# Autodesk Inventor assembly: Base_Rotation
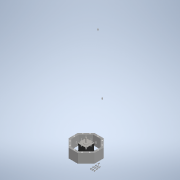
[picture p0: Inventor's stored thumbnail of the model, 180x180]
Saved by Autodesk Inventor 2022 (Build 260153000, 153)
## iProperties
Created: 2022-03-21
Part Number: Base_Rotation
Document SubType Name: Assembly
Designer: Mlees
Author: Mlees
## Documents named in this file (7)
- C:\Users\Mlees\Desktop\504Engineering\Project_0000\Designs\Design_1\Base_Rotation.iam
- C:\Users\Mlees\Desktop\504Engineering\Project_0000\Designs\Design_1\Created_Parts\Base_Mount.ipt
- C:\Users\Mlees\Desktop\504Engineering\Stepper-Servo_Based_Robotic_Arm\Designs\Version_8\Downloaded_Parts\Nema_17\Nema 17.ipt
- C:\Users\Mlees\Desktop\504Engineering\Project_0000\Designs\Design_1\Created_Parts\Base_Lid.ipt
- C:\Users\Mlees\Desktop\504Engineering\Project_0000\Designs\Design_1\Downloaded_Parts\Stainless Steel Pan Head Phillips Screws_m2.5x8mm.ipt
- C:\Users\Mlees\Desktop\504Engineering\Project_0000\Designs\Design_1\Downloaded_Parts\94180A333_Tapered Heat-Set Inserts for PlasticM3x6.4.ipt
- C:\Users\Mlees\Desktop\504Engineering\Project_0000\Designs\Design_1\Downloaded_Parts\90116A151_316 Stainless Steel Pan Head Phillips ScrewsM3x6mm.ipt
## Components (39 placed, 6 different names)
1. Base_Mount:1 — Mate:1, Rigid:1, Mate:2, Flush:1, Flush:2, Mate:27, Mate:28, Mate:29, Mate:30, Mate:31, Mate:32, Mate:33, Mate:35, Mate:36, Mate:37, Mate:39, Mate:40, Mate:41, Mate:42, Mate:43, Mate:44, Mate:45, Mate:46, Mate:47, Mate:48, Mate:49, Mate:50, Mate:53, Mate:54
2. Nema 17:1 — Mate:1, Rigid:1, Mate:3, Mate:5, Mate:6, Mate:7
3. Base_Lid:1 — Mate:2, Flush:1, Flush:2, Mate:4, Mate:8, Mate:9, Mate:10, Mate:11, Mate:12, Mate:13, Mate:14, Mate:15, Mate:16, Mate:17, Mate:18, Mate:19, Mate:20, Mate:21, Mate:22, Mate:23, Mate:24, Mate:25, Mate:26
4. Stainless Steel Pan Head Phillips Screws_m2.5x8mm:1 — Mate:3, Mate:4
5. Stainless Steel Pan Head Phillips Screws_m2.5x8mm:2 — Mate:5, Mate:8
6. Stainless Steel Pan Head Phillips Screws_m2.5x8mm:3 — Mate:6, Mate:10
7. Stainless Steel Pan Head Phillips Screws_m2.5x8mm:4 — Mate:7, Mate:9
8. Stainless Steel Pan Head Phillips Screws_m2.5x8mm:5 — Mate:15, Mate:20
9. Stainless Steel Pan Head Phillips Screws_m2.5x8mm:6 — Mate:14, Mate:19
10. Stainless Steel Pan Head Phillips Screws_m2.5x8mm:7 — Mate:16, Mate:26
11. Stainless Steel Pan Head Phillips Screws_m2.5x8mm:8 — Mate:13, Mate:23
12. Stainless Steel Pan Head Phillips Screws_m2.5x8mm:9 — Mate:18, Mate:21
13. Stainless Steel Pan Head Phillips Screws_m2.5x8mm:10 — Mate:17, Mate:22
14. Stainless Steel Pan Head Phillips Screws_m2.5x8mm:11 — Mate:12, Mate:24
15. Stainless Steel Pan Head Phillips Screws_m2.5x8mm:12 — Mate:11, Mate:25
16. 94180A333_Tapered Heat-Set Inserts for PlasticM3x6.4:1 — Mate:33, Mate:49
17. 94180A333_Tapered Heat-Set Inserts for PlasticM3x6.4:2 — Mate:35, Mate:46, Mate:52
18. 94180A333_Tapered Heat-Set Inserts for PlasticM3x6.4:3 — Mate:36, Mate:45, Mate:51
19. 94180A333_Tapered Heat-Set Inserts for PlasticM3x6.4:4 — Mate:47, Mate:54
20. 94180A333_Tapered Heat-Set Inserts for PlasticM3x6.4:5 — Mate:37, Mate:43
21. 94180A333_Tapered Heat-Set Inserts for PlasticM3x6.4:6 — Mate:42, Mate:53
22. 94180A333_Tapered Heat-Set Inserts for PlasticM3x6.4:7 — Mate:32, Mate:50
23. 94180A333_Tapered Heat-Set Inserts for PlasticM3x6.4:8 — Mate:31, Mate:48
24. 94180A333_Tapered Heat-Set Inserts for PlasticM3x6.4:9 — Mate:30, Mate:44
25. 94180A333_Tapered Heat-Set Inserts for PlasticM3x6.4:10 — Mate:29, Mate:39
26. 94180A333_Tapered Heat-Set Inserts for PlasticM3x6.4:11 — Mate:27, Mate:41
27. 94180A333_Tapered Heat-Set Inserts for PlasticM3x6.4:12 — Mate:28, Mate:40
28. 90116A151_316 Stainless Steel Pan Head Phillips ScrewsM3x6mm:1
29. 90116A151_316 Stainless Steel Pan Head Phillips ScrewsM3x6mm:2
30. 90116A151_316 Stainless Steel Pan Head Phillips ScrewsM3x6mm:3
31. 90116A151_316 Stainless Steel Pan Head Phillips ScrewsM3x6mm:4
32. 90116A151_316 Stainless Steel Pan Head Phillips ScrewsM3x6mm:5 — Mate:52
33. 90116A151_316 Stainless Steel Pan Head Phillips ScrewsM3x6mm:6 — Mate:51
34. 90116A151_316 Stainless Steel Pan Head Phillips ScrewsM3x6mm:7
35. 90116A151_316 Stainless Steel Pan Head Phillips ScrewsM3x6mm:8
36. 90116A151_316 Stainless Steel Pan Head Phillips ScrewsM3x6mm:9
37. 90116A151_316 Stainless Steel Pan Head Phillips ScrewsM3x6mm:10
38. 90116A151_316 Stainless Steel Pan Head Phillips ScrewsM3x6mm:11
39. 90116A151_316 Stainless Steel Pan Head Phillips ScrewsM3x6mm:12
## Relationships (55: Mate 52, Flush 2, WeldJoint 1)
- Mate:1: Base_Mount:1 ↔ Nema 17:1
- Rigid:1 [WeldJoint]: Base_Mount:1 ↔ Nema 17:1
- Mate:2: Base_Mount:1 ↔ Base_Lid:1
- Flush:1: Base_Mount:1 ↔ Base_Lid:1
- Flush:2: Base_Mount:1 ↔ Base_Lid:1
- Mate:3: Nema 17:1 ↔ Stainless Steel Pan Head Phillips Screws_m2.5x8mm:1
- Mate:4: Base_Lid:1 ↔ Stainless Steel Pan Head Phillips Screws_m2.5x8mm:1
- Mate:5: Nema 17:1 ↔ Stainless Steel Pan Head Phillips Screws_m2.5x8mm:2
- Mate:6: Nema 17:1 ↔ Stainless Steel Pan Head Phillips Screws_m2.5x8mm:3
- Mate:7: Nema 17:1 ↔ Stainless Steel Pan Head Phillips Screws_m2.5x8mm:4
- Mate:8: Base_Lid:1 ↔ Stainless Steel Pan Head Phillips Screws_m2.5x8mm:2
- Mate:9: Base_Lid:1 ↔ Stainless Steel Pan Head Phillips Screws_m2.5x8mm:4
- Mate:10: Base_Lid:1 ↔ Stainless Steel Pan Head Phillips Screws_m2.5x8mm:3
- Mate:11: Base_Lid:1 ↔ Stainless Steel Pan Head Phillips Screws_m2.5x8mm:12
- Mate:12: Base_Lid:1 ↔ Stainless Steel Pan Head Phillips Screws_m2.5x8mm:11
- Mate:13: Base_Lid:1 ↔ Stainless Steel Pan Head Phillips Screws_m2.5x8mm:8
- Mate:14: Base_Lid:1 ↔ Stainless Steel Pan Head Phillips Screws_m2.5x8mm:6
- Mate:15: Base_Lid:1 ↔ Stainless Steel Pan Head Phillips Screws_m2.5x8mm:5
- Mate:16: Base_Lid:1 ↔ Stainless Steel Pan Head Phillips Screws_m2.5x8mm:7
- Mate:17: Base_Lid:1 ↔ Stainless Steel Pan Head Phillips Screws_m2.5x8mm:10
- Mate:18: Base_Lid:1 ↔ Stainless Steel Pan Head Phillips Screws_m2.5x8mm:9
- Mate:19: Base_Lid:1 ↔ Stainless Steel Pan Head Phillips Screws_m2.5x8mm:6
- Mate:20: Base_Lid:1 ↔ Stainless Steel Pan Head Phillips Screws_m2.5x8mm:5
- Mate:21: Base_Lid:1 ↔ Stainless Steel Pan Head Phillips Screws_m2.5x8mm:9
- Mate:22: Base_Lid:1 ↔ Stainless Steel Pan Head Phillips Screws_m2.5x8mm:10
- Mate:23: Base_Lid:1 ↔ Stainless Steel Pan Head Phillips Screws_m2.5x8mm:8
- Mate:24: Base_Lid:1 ↔ Stainless Steel Pan Head Phillips Screws_m2.5x8mm:11
- Mate:25: Base_Lid:1 ↔ Stainless Steel Pan Head Phillips Screws_m2.5x8mm:12
- Mate:26: Base_Lid:1 ↔ Stainless Steel Pan Head Phillips Screws_m2.5x8mm:7
- Mate:27: Base_Mount:1 ↔ 94180A333_Tapered Heat-Set Inserts for PlasticM3x6.4:11
- Mate:28: Base_Mount:1 ↔ 94180A333_Tapered Heat-Set Inserts for PlasticM3x6.4:12
- Mate:29: Base_Mount:1 ↔ 94180A333_Tapered Heat-Set Inserts for PlasticM3x6.4:10
- Mate:30: Base_Mount:1 ↔ 94180A333_Tapered Heat-Set Inserts for PlasticM3x6.4:9
- Mate:31: Base_Mount:1 ↔ 94180A333_Tapered Heat-Set Inserts for PlasticM3x6.4:8
- Mate:32: Base_Mount:1 ↔ 94180A333_Tapered Heat-Set Inserts for PlasticM3x6.4:7
- Mate:33: Base_Mount:1 ↔ 94180A333_Tapered Heat-Set Inserts for PlasticM3x6.4:1
- Mate:35: Base_Mount:1 ↔ 94180A333_Tapered Heat-Set Inserts for PlasticM3x6.4:2
- Mate:36: Base_Mount:1 ↔ 94180A333_Tapered Heat-Set Inserts for PlasticM3x6.4:3
- Mate:37: Base_Mount:1 ↔ 94180A333_Tapered Heat-Set Inserts for PlasticM3x6.4:5
- Mate:39: Base_Mount:1 ↔ 94180A333_Tapered Heat-Set Inserts for PlasticM3x6.4:10
- Mate:40: Base_Mount:1 ↔ 94180A333_Tapered Heat-Set Inserts for PlasticM3x6.4:12
- Mate:41: Base_Mount:1 ↔ 94180A333_Tapered Heat-Set Inserts for PlasticM3x6.4:11
- Mate:42: Base_Mount:1 ↔ 94180A333_Tapered Heat-Set Inserts for PlasticM3x6.4:6
- Mate:43: Base_Mount:1 ↔ 94180A333_Tapered Heat-Set Inserts for PlasticM3x6.4:5
- Mate:44: Base_Mount:1 ↔ 94180A333_Tapered Heat-Set Inserts for PlasticM3x6.4:9
- Mate:45: Base_Mount:1 ↔ 94180A333_Tapered Heat-Set Inserts for PlasticM3x6.4:3
- Mate:46: Base_Mount:1 ↔ 94180A333_Tapered Heat-Set Inserts for PlasticM3x6.4:2
- Mate:47: Base_Mount:1 ↔ 94180A333_Tapered Heat-Set Inserts for PlasticM3x6.4:4
- Mate:48: Base_Mount:1 ↔ 94180A333_Tapered Heat-Set Inserts for PlasticM3x6.4:8
- Mate:49: Base_Mount:1 ↔ 94180A333_Tapered Heat-Set Inserts for PlasticM3x6.4:1
- Mate:50: Base_Mount:1 ↔ 94180A333_Tapered Heat-Set Inserts for PlasticM3x6.4:7
- Mate:51: 94180A333_Tapered Heat-Set Inserts for PlasticM3x6.4:3 ↔ 90116A151_316 Stainless Steel Pan Head Phillips ScrewsM3x6mm:6
- Mate:52: 94180A333_Tapered Heat-Set Inserts for PlasticM3x6.4:2 ↔ 90116A151_316 Stainless Steel Pan Head Phillips ScrewsM3x6mm:5
- Mate:53: Base_Mount:1 ↔ 94180A333_Tapered Heat-Set Inserts for PlasticM3x6.4:6
- Mate:54: Base_Mount:1 ↔ 94180A333_Tapered Heat-Set Inserts for PlasticM3x6.4:4
